# Autodesk Inventor assembly: 217-2615 wUS Digital Encoder.20121204
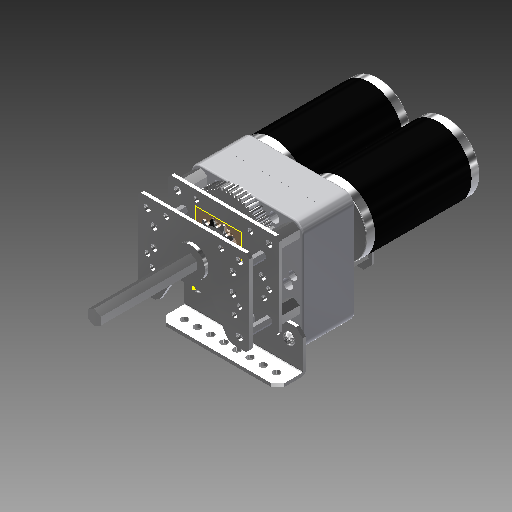
[picture p0: Inventor's stored thumbnail of the model, 512x512]
Saved by Autodesk Inventor 2017 (Build 210142000, 142)
## iProperties
Company: Microsoft
Created: 2012-12-05
Part Number: 217-2615 wUS Digital Encoder.20121204
Description: STEP AP203
Document SubType Name: Assembly
Designer: solomon
Mass: 2876.4 g
Surface Area: 4224.13 cm^2
Volume: 1237.93 cm^3
Density: 2.32355 g/cm^3
Sending System: SolidWorks 2012
Preprocessor: SwSTEP 2.0
Title: Vex DS BS
Author: svradm
Revision Number: ANY
## Documents named in this file (46)
- C:\Users\solomon\Documents\Inventor\2012bot\COTS\Gearboxes\Vex\2 CIM Ball Shifter\217-2615 wUS Digital Encoder.20121204.iam
- C:\Users\solomon\Documents\Inventor\2012bot\COTS\Gearboxes\Vex\2 CIM Ball Shifter\217-2733.ipt
- C:\Users\solomon\Documents\Inventor\2012bot\COTS\Gearboxes\Vex\2 CIM Ball Shifter\217-2731.ipt
- C:\Users\solomon\Documents\Inventor\2012bot\COTS\Gearboxes\Vex\2 CIM Ball Shifter\217-2789.ipt
- C:\Users\solomon\Documents\Inventor\2012bot\COTS\Gearboxes\Vex\2 CIM Ball Shifter\217-2428-027 Rev1_97414A630.ipt
- C:\Users\solomon\Documents\Inventor\2012bot\COTS\Gearboxes\Vex\2 CIM Ball Shifter\217-2788_57155K375.ipt
- C:\Users\solomon\Documents\Inventor\2012bot\COTS\Gearboxes\Vex\2 CIM Ball Shifter\217-2428-011 Rev2 .ipt
- C:\Users\solomon\Documents\Inventor\2012bot\COTS\Gearboxes\Vex\2 CIM Ball Shifter\217-2428-012 Rev1.ipt
- C:\Users\solomon\Documents\Inventor\2012bot\COTS\Gearboxes\Vex\2 CIM Ball Shifter\217-2428-005 Rev1.ipt
- C:\Users\solomon\Documents\Inventor\2012bot\COTS\Gearboxes\Vex\2 CIM Ball Shifter\SCREW-B-440-0250_91306A311.ipt
- C:\Users\solomon\Documents\Inventor\2012bot\COTS\Gearboxes\Vex\2 CIM Ball Shifter\SCREW-832-0375.ipt
- C:\Users\solomon\Documents\Inventor\2012bot\COTS\Gearboxes\Vex\2 CIM Ball Shifter\217-2428-016 Rev2_Spur01.ipt
- C:\Users\solomon\Documents\Inventor\2012bot\COTS\Gearboxes\Vex\2 CIM Ball Shifter\217-2428-017 Rev2.ipt
- C:\Users\solomon\Documents\Inventor\2012bot\COTS\Gearboxes\Vex\2 CIM Ball Shifter\217-2428-018 Rev2.ipt
- C:\Users\solomon\Documents\Inventor\2012bot\COTS\Gearboxes\Vex\2 CIM Ball Shifter\217-2428-009 Rev1.ipt
- C:\Users\solomon\Documents\Inventor\2012bot\COTS\Gearboxes\Vex\2 CIM Ball Shifter\SCREW-832-0250.ipt
- C:\Users\solomon\Documents\Inventor\2012bot\COTS\Gearboxes\Vex\2 CIM Ball Shifter\PINL-0250-1125-S.ipt
- C:\Users\solomon\Documents\Inventor\2012bot\COTS\Gearboxes\Vex\2 CIM Ball Shifter\217-2614-001_12t.ipt
- C:\Users\solomon\Documents\Inventor\2012bot\COTS\Gearboxes\Vex\2 CIM Ball Shifter\217-2761-001 rev1.ipt
- C:\Users\solomon\Documents\Inventor\2012bot\COTS\Gearboxes\Vex\2 CIM Ball Shifter\217-2428-001 Rev1.ipt
- C:\Users\solomon\Documents\Inventor\2012bot\COTS\Gearboxes\Vex\2 CIM Ball Shifter\217-2428-002 Rev1.ipt
- C:\Users\solomon\Documents\Inventor\2012bot\COTS\Gearboxes\Vex\2 CIM Ball Shifter\217-2703-001.ipt
- C:\Users\solomon\Documents\Inventor\2012bot\COTS\Gearboxes\Vex\2 CIM Ball Shifter\217-2707-001_40t.ipt
- C:\Users\solomon\Documents\Inventor\2012bot\COTS\Gearboxes\Vex\2 CIM Ball Shifter\SBS1_SBS0832-1750SS.ipt
- C:\Users\solomon\Documents\Inventor\2012bot\COTS\Gearboxes\Vex\2 CIM Ball Shifter\Nylock Nut_NNY2520-ZC.ipt
- C:\Users\solomon\Documents\Inventor\2012bot\COTS\Gearboxes\Vex\2 CIM Ball Shifter\217-2428-004 Rev3.ipt
- C:\Users\solomon\Documents\Inventor\2012bot\COTS\Gearboxes\Vex\2 CIM Ball Shifter\217-2428-021 Rev1.ipt
- C:\Users\solomon\Documents\Inventor\2012bot\COTS\Gearboxes\Vex\2 CIM Ball Shifter\217-2428-029 Rev1.ipt
- C:\Users\solomon\Documents\Inventor\2012bot\COTS\Gearboxes\Vex\2 CIM Ball Shifter\Nylock 8-32.ipt
- C:\Users\solomon\Documents\Inventor\2012bot\COTS\Gearboxes\Vex\2 CIM Ball Shifter\217-2793-001 Rev1.iam
- C:\Users\solomon\Documents\Inventor\2012bot\COTS\Gearboxes\Vex\2 CIM Ball Shifter\217-2000.ipt
- C:\Users\solomon\Documents\Inventor\2012bot\COTS\Gearboxes\Vex\2 CIM Ball Shifter\E4P-X-250-X-D-D-D-X.ipt
- C:\Users\solomon\Documents\Inventor\2012bot\COTS\Gearboxes\Vex\2 CIM Ball Shifter\217-2617-003 Rev1.ipt
- C:\Users\solomon\Documents\Inventor\2012bot\COTS\Gearboxes\Vex\2 CIM Ball Shifter\217-2743.ipt
- C:\Users\solomon\Documents\Inventor\2012bot\COTS\Gearboxes\Vex\2 CIM Ball Shifter\217-2734.ipt
- C:\Users\solomon\Documents\Inventor\2012bot\COTS\Gearboxes\Vex\2 CIM Ball Shifter\217-2704-001_30.ipt
- C:\Users\solomon\Documents\Inventor\2012bot\COTS\Gearboxes\Vex\2 CIM Ball Shifter\217-2714-001_60t.ipt
- C:\Users\solomon\Documents\Inventor\2012bot\COTS\Gearboxes\Vex\2 CIM Ball Shifter\217-2617-001 Rev4.ipt
- C:\Users\solomon\Documents\Inventor\2012bot\COTS\Gearboxes\Vex\2 CIM Ball Shifter\217-2617-002 Rev1_91780A359.ipt
- C:\Users\solomon\Documents\Inventor\2012bot\COTS\Gearboxes\Vex\2 CIM Ball Shifter\217-2617-004 Rev1_97431A340_grv.ipt
- C:\Users\solomon\Documents\Inventor\2012bot\COTS\Gearboxes\Vex\2 CIM Ball Shifter\SBS1_SBS2520-1750.ipt
- C:\Users\solomon\Documents\Inventor\2012bot\COTS\Gearboxes\Vex\2 CIM Ball Shifter\217-2778-001 Rev2_NCQ8A075-050M.iam
- C:\Users\solomon\Documents\Inventor\2012bot\COTS\Gearboxes\Vex\2 CIM Ball Shifter\217-2428-024 Rev2.ipt
- C:\Users\solomon\Documents\Inventor\2012bot\COTS\Gearboxes\Vex\2 CIM Ball Shifter\SBS1_SBS2520-2000ZC.ipt
- C:\Users\solomon\Documents\Inventor\2012bot\COTS\Structure\VersaFrame\West Cost Bearing Blocks\217-2658.20121204.ipt
- C:\Users\solomon\Documents\Inventor\2012bot\COTS\Hardware\275-1016-001.ipt
## Components (78 placed, 75 different names)
1. 217-2733_1
2. 217-2733_2
3. 217-2731_3
4. 217-2789_4
5. 217-2428-027 Rev1_97414A630_5
6. 217-2788_57155K375_6
7. 217-2428-011 Rev2 _7
8. 217-2428-012 Rev1_8
9. 217-2428-027 Rev1_97414A630_9
10. 217-2428-005 Rev1_10
11. 217-2428-005 Rev1_11
12. SCREW-B-440-0250_91306A311_12
13. SCREW-B-440-0250_91306A311_13
14. SCREW-B-440-0250_91306A311_14
15. SCREW-832-0375_15
16. SCREW-832-0375_16
17. SCREW-832-0375_17
18. SCREW-832-0375_18
19. 217-2428-016 Rev2_Spur01_19
20. 217-2428-017 Rev2_20
21. 217-2428-018 Rev2_21
22. 217-2788_57155K375_22
23. 217-2788_57155K375_23
24. 217-2428-009 Rev1_24
25. 217-2428-009 Rev1_25
26. SCREW-832-0250_26
27. SCREW-832-0375_27
28. SCREW-832-0375_28
29. SCREW-832-0250_29
30. PINL-0250-1125-S_30
31. 217-2614-001_12t_31
32. 217-2761-001 rev1_32
33. 217-2761-001 rev1_33
34. 217-2614-001_12t_34
35. 217-2428-001 Rev1_35
36. 217-2428-002 Rev1_36
37. 217-2703-001_37
38. 217-2707-001_40t_38
39. SBS1_SBS0832-1750SS_39
40. SBS1_SBS0832-1750SS_40
41. Nylock Nut_NNY2520-ZC_41
42. 217-2428-004 Rev3_42
43. 217-2428-021 Rev1_43
44. 217-2428-029 Rev1_44
45. Nylock 8-32_45
46. Nylock 8-32_46
47. 217-2793-001 Rev1_47 [sub-assembly]
48. 217-2000_48
49. 217-2000_49
50. E4P-X-250-X-D-D-D-X_50
51. 217-2617-003 Rev1_51 — Angle:1, Mate:3
52. 217-2743_52
53. 217-2734_53 — Mate:1
54. 217-2704-001_30_54
55. 217-2714-001_60t_55
56. 217-2617-001 Rev4_56 — Mate:7, Mate:8, Mate:9, Mate:10
57. 217-2617-002 Rev1_91780A359_57
58. 217-2617-002 Rev1_91780A359_58
59. 217-2617-002 Rev1_91780A359_59
60. 217-2617-002 Rev1_91780A359_60
61. 217-2617-004 Rev1_97431A340_grv_61
62. 217-2617-004 Rev1_97431A340_grv_62
63. SBS1_SBS2520-1750_63
64. SBS1_SBS2520-1750_64
65. SBS1_SBS2520-1750_65
66. SBS1_SBS2520-1750_66
67. 217-2778-001 Rev2_NCQ8A075-050M_71 [sub-assembly]
68. 217-2428-024 Rev2_72
69. Nylock Nut_NNY2520-ZC_73
70. SBS1_SBS2520-2000ZC_74
71. SBS1_SBS2520-2000ZC_75
72. 217-2658.20121204:1 — Angle:1, Mate:1, Mate:2
73. 217-2617-001 Rev4:2 — Mate:4, Angle:2, Angle:3, Mate:11
74. 217-2734:2 — Mate:2, Mate:3, Mate:4
75. 275-1016-001:3 — Mate:7
76. 275-1016-001:4 — Mate:8
77. 275-1016-001:5 — Angle:3, Mate:9, Mate:11
78. 275-1016-001:6 — Angle:2, Mate:10
## Relationships (12: Mate 9, Angle 3)
- Angle:1 (0 deg): 217-2617-003 Rev1_51 ↔ 217-2658.20121204:1
- Mate:1: 217-2734_53 ↔ 217-2658.20121204:1
- Mate:2: 217-2658.20121204:1 ↔ 217-2734:2
- Mate:3: 217-2617-003 Rev1_51 ↔ 217-2734:2
- Mate:4: 217-2617-001 Rev4:2 ↔ 217-2734:2
- Mate:7: 217-2617-001 Rev4_56 ↔ 275-1016-001:3
- Mate:8: 217-2617-001 Rev4_56 ↔ 275-1016-001:4
- Angle:2 (0 deg): 217-2617-001 Rev4:2 ↔ 275-1016-001:6
- Angle:3 (0 deg): 217-2617-001 Rev4:2 ↔ 275-1016-001:5
- Mate:9: 217-2617-001 Rev4_56 ↔ 275-1016-001:5
- Mate:10: 217-2617-001 Rev4_56 ↔ 275-1016-001:6
- Mate:11: 217-2617-001 Rev4:2 ↔ 275-1016-001:5
